# Autodesk Inventor assembly: Additional_Building
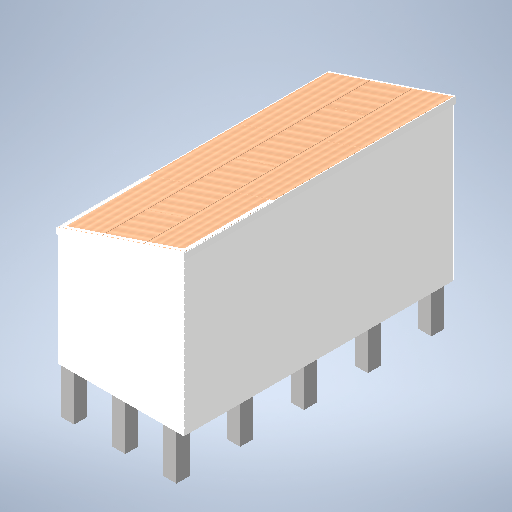
[picture p0: Inventor's stored thumbnail of the model, 512x512]
Saved by Autodesk Inventor 2025 (Build 290162010, 162A)
## iProperties
Created: 2024-08-02
Part Number: Additional_Building
Document SubType Name: Assembly
Designer: Tom
Author: Tom
## Documents named in this file (52)
- C:\Users\Tom\Documents\Inventor\Mobility\Additional_Building\Additional_Building.iam
- C:\Users\Tom\Documents\Inventor\Mobility\Additional_Building\Grid_Of_Piers.iam
- C:\Users\Tom\Documents\Inventor\Mobility\Additional_Building\Floor_System.iam
- C:\Users\Tom\Documents\Inventor\Mobility\Additional_Building\Walls.iam
- C:\Users\Tom\Documents\Inventor\Mobility\Additional_Building\Truss.iam
- C:\Users\Tom\Documents\Inventor\Mobility\Additional_Building\OSB_For_Walls_With_Dimensions_48_x_96_Inches.ipt
- C:\Users\Tom\Documents\Inventor\Mobility\Additional_Building\OSB_For_Walls_With_Dimensions_48_x_48_Inches.ipt
- C:\Users\Tom\Documents\Inventor\Mobility\Additional_Building\OSB_For_Roof_With_Dimensions_96_x_48.ipt
- C:\Users\Tom\Documents\Inventor\Mobility\Additional_Building\OSB_For_Walls_With_Dimensions_25.5_x_96_Inches.ipt
- C:\Users\Tom\Documents\Inventor\Mobility\Additional_Building\Subfascia_With_Dimensions_4.023_x_13.75_Inches.ipt
- C:\Users\Tom\Documents\Inventor\Mobility\Additional_Building\Subfascia_With_Dimensions_4.023_x_14.5_Inches.ipt
- C:\Users\Tom\Documents\Inventor\Mobility\Additional_Building\DensGlass_With_Dimensions_36.5_x_48_Inches.ipt
- C:\Users\Tom\Documents\Inventor\Mobility\Additional_Building\DensGlass_With_Dimensions_48_x_96_Inches.ipt
- C:\Users\Tom\Documents\Inventor\Mobility\Additional_Building\DensGlass_With_Dimensions_48_x_84.5_Inches.ipt
- C:\Users\Tom\Documents\Inventor\Mobility\Additional_Building\DensGlass_With_Dimensions_60.75_x_12_Inches.ipt
- C:\Users\Tom\Documents\Inventor\Mobility\Additional_Building\DensGlass_With_Dimensions_36.5_x_25.5_Inches.ipt
- C:\Users\Tom\Documents\Inventor\Mobility\Additional_Building\DensGlass_With_Dimensions_25.5_x_96_Inches.ipt
- C:\Users\Tom\Documents\Inventor\Mobility\Additional_Building\Siding_For_Back_Wall.iam
- C:\Users\Tom\Documents\Inventor\Mobility\Additional_Building\Fascia_For_Back.ipt
- C:\Users\Tom\Documents\Inventor\Mobility\Additional_Building\OSB_For_Side_And_Back.ipt
- C:\Users\Tom\Documents\Inventor\Mobility\Additional_Building\OSB_For_Roof_With_Dimensions_48_x_48.ipt
- C:\Users\Tom\Documents\Inventor\Mobility\Additional_Building\OSB_For_Roof_With_Dimensions_46.416_x_96.ipt
- C:\Users\Tom\Documents\Inventor\Mobility\Additional_Building\Stud_Between_Top_Plate_And_Rafter_1.ipt
- C:\Users\Tom\Documents\Inventor\Mobility\Additional_Building\Stud_Between_Top_Plate_And_Rafter_2.ipt
- C:\Users\Tom\Documents\Inventor\Mobility\Additional_Building\Stud_Between_Top_Plate_And_Rafter_3.ipt
- C:\Users\Tom\Documents\Inventor\Mobility\Additional_Building\Stud_Between_Top_Plate_And_Rafter_4.ipt
- C:\Users\Tom\Documents\Inventor\Mobility\Additional_Building\Stud_Between_Top_Plate_And_Rafter_5.ipt
- C:\Users\Tom\Documents\Inventor\Mobility\Additional_Building\Stud_Between_Top_Plate_And_Rafter_6.ipt
- C:\Users\Tom\Documents\Inventor\Mobility\Additional_Building\Stud_Between_Top_Plate_And_Rafter_7.ipt
- C:\Users\Tom\Documents\Inventor\Mobility\Additional_Building\Stud_Between_Top_Plate_And_Rafter_8.ipt
- C:\Users\Tom\Documents\Inventor\Mobility\Additional_Building\Stud_Between_Top_Plate_And_Rafter_9.ipt
- C:\Users\Tom\Documents\Inventor\Mobility\Additional_Building\Stud_With_Height_41.707_Inches.ipt
- C:\Users\Tom\Documents\Inventor\Mobility\Additional_Building\Support_For_Ceiling.ipt
- C:\Users\Tom\Documents\Inventor\Mobility\Additional_Building\OSB_For_Side_And_Front.ipt
- C:\Users\Tom\Documents\Inventor\Mobility\Additional_Building\OSB_For_Side_And_Top.ipt
- C:\Users\Tom\Documents\Inventor\Mobility\Additional_Building\Subfascia_With_Dimensions_5.798_x_13.75_Inches.ipt
- C:\Users\Tom\Documents\Inventor\Mobility\Additional_Building\Subfascia_With_Dimensions_5.798_x_14.5_Inches.ipt
- C:\Users\Tom\Documents\Inventor\Mobility\Additional_Building\OSB_For_Walls_With_Dimensions_20.794_x_48_Inches.ipt
- C:\Users\Tom\Documents\Inventor\Mobility\Additional_Building\OSB_For_Walls_With_Dimensions_20.794_x_96_Inches.ipt
- C:\Users\Tom\Documents\Inventor\Mobility\Additional_Building\Siding_For_Front_Wall.iam
- C:\Users\Tom\Documents\Inventor\Mobility\Additional_Building\Fascia_For_Front.ipt
- C:\Users\Tom\Documents\Inventor\Mobility\Additional_Building\OSB_For_Walls_With_Dimensions_48_x_85_Inches.ipt
- C:\Users\Tom\Documents\Inventor\Mobility\Additional_Building\OSB_For_Walls_With_Dimensions_37_x_48_Inches.ipt
- C:\Users\Tom\Documents\Inventor\Mobility\Additional_Building\Fascia_For_Side.ipt
- C:\Users\Tom\Documents\Inventor\Mobility\Additional_Building\Drip_Edge_For_Back.ipt
- C:\Users\Tom\Documents\Inventor\Mobility\Additional_Building\OSB_For_Rear_Roof.ipt
- C:\Users\Tom\Documents\Inventor\Mobility\Additional_Building\Siding_For_Left_Wall.iam
- C:\Users\Tom\Documents\Inventor\Mobility\Additional_Building\Siding_For_Right_Wall.iam
- C:\Users\Tom\Documents\Inventor\Mobility\Additional_Building\Drip_Edge_For_Front.ipt
- C:\Users\Tom\Documents\Inventor\Mobility\Additional_Building\Drip_Edge_For_Side.ipt
- C:\Users\Tom\Documents\Inventor\Mobility\Additional_Building\Underlayment_For_Side.ipt
- C:\Users\Tom\Documents\Inventor\Mobility\Additional_Building\Underlayment_For_Front.ipt
## Components (179 placed, 51 different names)
1. Grid_Of_Piers:1 [sub-assembly] — Mate:1, Flush:1, Mate:2
2. Floor_System:1 [sub-assembly] — Mate:1, Flush:1, Mate:2, Mate:3, Flush:2, Flush:3, Flush:15, Flush:16, Flush:29, Flush:30, Flush:31, Flush:33
3. Walls:1 [sub-assembly] — Mate:3, Flush:2, Flush:3, Flush:4, Flush:5, Mate:4, Flush:7, Mate:5, Mate:9, Mate:10, Flush:17, Mate:12, Mate:15, Mate:18, Mate:68, Flush:48, Flush:49, Mate:69, Flush:50, Flush:51, Mate:70, Flush:52, Flush:53, Mate:71, Flush:54, Flush:55, Mate:72, Flush:56, Flush:57, Mate:73, Flush:58, Flush:59, Mate:74, Flush:60, Flush:61, Mate:75, Flush:62, Flush:63, Mate:76, Flush:64, Mate:78, Mate:90, Mate:113, Mate:116, Mate:119, Mate:121
4. Subfascia_With_Dimensions_4.023_x_13.75_Inches:1 — Mate:21, Flush:22, Flush:23
5. Subfascia_With_Dimensions_4.023_x_13.75_Inches:2 — Flush:26, Mate:23, Flush:27, Flush:39
6. DensGlass_With_Dimensions_36.5_x_48_Inches:1 — Mate:24, Flush:28, Flush:29, Mate:26
7. DensGlass_With_Dimensions_36.5_x_48_Inches:2 — Mate:27, Mate:28, Flush:31
8. DensGlass_With_Dimensions_48_x_84.5_Inches:1 — Mate:29, Flush:32, Mate:30, Mate:32, Mate:38, Mate:41, Mate:44
9. DensGlass_With_Dimensions_48_x_96_Inches:3 — Mate:31, Mate:32, Mate:33, Mate:35
10. DensGlass_With_Dimensions_48_x_84.5_Inches:2 — Mate:34, Mate:35, Mate:36, Mate:47
11. DensGlass_With_Dimensions_36.5_x_25.5_Inches:1 — Mate:39, Mate:40, Mate:41, Mate:43
12. DensGlass_With_Dimensions_36.5_x_25.5_Inches:2 — Mate:45, Mate:46, Mate:47
13. Siding_For_Back_Wall:1 [sub-assembly] — Mate:48, Flush:34, Flush:35
14. Underlayment_For_Front:1 — Mate:146, Flush:126, Mate:147
15. Siding_For_Front_Wall:1 [sub-assembly] — Flush:93, Flush:94, Mate:108
16. Underlayment_For_Side:1 — Mate:144, Flush:122, Flush:123
17. Siding_For_Left_Wall:1 [sub-assembly] — Mate:133, Flush:117, Mate:134
18. Fascia_For_Side:1 — Mate:126, Flush:105, Flush:108, Mate:141, Mate:142
19. Underlayment_For_Side:2 — Flush:124, Mate:145, Flush:125, Flush:126
20. Siding_For_Right_Wall:1 [sub-assembly] — Mate:135, Mate:136, Flush:118
21. Fascia_For_Side:2 — Mate:127, Flush:107, Flush:108
22. Drip_Edge_For_Side:1 — Mate:140, Mate:141, Flush:120
23. Drip_Edge_For_Back:1 — Flush:109, Mate:128, Mate:137
24. Drip_Edge_For_Front:1 — Mate:138, Flush:119
25. Truss:1 [sub-assembly] — Flush:6, Mate:23, Flush:27, Mate:50, Mate:56, Mate:77, Mate:79, Flush:65, Flush:67, Flush:69, Flush:71, Flush:73, Flush:75, Flush:77, Flush:79, Flush:81, Mate:92, Mate:96, Mate:109, Flush:104, Flush:115, Mate:132, Flush:116, Mate:153
26. Truss:2 [sub-assembly] — Flush:4, Flush:5, Mate:4, Mate:20, Mate:101, Flush:91, Mate:103, Flush:92, Flush:124, Mate:147, Flush:127
27. Truss:3 [sub-assembly] — Flush:6, Flush:7, Mate:5, Flush:26, Mate:81, Mate:82, Mate:83, Mate:84, Mate:85, Mate:86, Mate:87, Mate:88, Mate:89, Mate:91, Flush:82, Mate:99, Flush:87, Flush:88
28. Truss:4 [sub-assembly] — Mate:100, Flush:89, Flush:90
29. Truss:5 [sub-assembly]
30. Truss:6 [sub-assembly]
31. Truss:7 [sub-assembly]
32. Truss:8 [sub-assembly]
33. Truss:9 [sub-assembly]
34. Truss:10 [sub-assembly]
35. Truss:11 [sub-assembly]
36. Truss:12 [sub-assembly]
37. Truss:13 [sub-assembly]
38. Truss:14 [sub-assembly]
39. Truss:15 [sub-assembly] — Mate:63
40. Truss:16 [sub-assembly] — Mate:105
41. Truss:17 [sub-assembly]
42. Truss:18 [sub-assembly] — Mate:22, Flush:25
43. Truss:19 [sub-assembly] — Mate:21, Flush:22, Flush:23, Flush:24, Mate:149
44. OSB_For_Walls_With_Dimensions_25.5_x_96_Inches:1 — Mate:18, Flush:18, Mate:20, Mate:39
45. OSB_For_Walls_With_Dimensions_25.5_x_96_Inches:2 — Mate:42
46. OSB_For_Walls_With_Dimensions_25.5_x_96_Inches:3 — Mate:45
47. OSB_For_Walls_With_Dimensions_48_x_48_Inches:2 — Mate:15, Mate:16, Mate:17, Mate:29, Flush:32
48. OSB_For_Walls_With_Dimensions_48_x_48_Inches:1 — Mate:10, Mate:11, Flush:17, Mate:13, Mate:34
49. OSB_For_Walls_With_Dimensions_48_x_48_Inches:3 — Mate:102
50. OSB_For_Walls_With_Dimensions_48_x_48_Inches:4
51. OSB_For_Walls_With_Dimensions_48_x_96_Inches:13 — Mate:101, Mate:102, Flush:91, Mate:104, Mate:108
52. OSB_For_Walls_With_Dimensions_48_x_96_Inches:14 — Mate:106
53. OSB_For_Walls_With_Dimensions_48_x_96_Inches:15 — Mate:146
54. OSB_For_Walls_With_Dimensions_20.794_x_96_Inches:1 — Mate:105, Mate:106, Mate:107
55. OSB_For_Walls_With_Dimensions_20.794_x_96_Inches:2
56. OSB_For_Walls_With_Dimensions_20.794_x_48_Inches:1 — Mate:103, Mate:104, Flush:92, Mate:107
57. OSB_For_Walls_With_Dimensions_20.794_x_48_Inches:2
58. Subfascia_With_Dimensions_4.023_x_14.5_Inches:1 — Flush:24, Mate:22, Flush:25
59. Subfascia_With_Dimensions_4.023_x_14.5_Inches:2
60. Subfascia_With_Dimensions_4.023_x_14.5_Inches:3
61. Subfascia_With_Dimensions_4.023_x_14.5_Inches:4
62. Subfascia_With_Dimensions_4.023_x_14.5_Inches:5
63. Subfascia_With_Dimensions_4.023_x_14.5_Inches:6
64. Subfascia_With_Dimensions_4.023_x_14.5_Inches:7
65. Subfascia_With_Dimensions_4.023_x_14.5_Inches:8
66. Subfascia_With_Dimensions_4.023_x_14.5_Inches:9
67. Subfascia_With_Dimensions_4.023_x_14.5_Inches:10
68. Subfascia_With_Dimensions_4.023_x_14.5_Inches:11
69. Subfascia_With_Dimensions_4.023_x_14.5_Inches:12
70. Subfascia_With_Dimensions_4.023_x_14.5_Inches:13
71. Subfascia_With_Dimensions_4.023_x_14.5_Inches:14
72. Subfascia_With_Dimensions_4.023_x_14.5_Inches:15
73. Subfascia_With_Dimensions_4.023_x_14.5_Inches:16
74. DensGlass_With_Dimensions_48_x_96_Inches:1 — Mate:25, Mate:26, Flush:30, Mate:30, Mate:33
75. DensGlass_With_Dimensions_48_x_96_Inches:2 — Mate:28, Mate:36
76. DensGlass_With_Dimensions_60.75_x_12_Inches:1 — Mate:37, Mate:38, Flush:33
77. DensGlass_With_Dimensions_60.75_x_12_Inches:2 — Mate:48, Flush:34, Flush:35
78. DensGlass_With_Dimensions_60.75_x_12_Inches:3 — Mate:40
79. DensGlass_With_Dimensions_60.75_x_12_Inches:4 — Mate:57, Mate:115
80. DensGlass_With_Dimensions_25.5_x_96_Inches:1 — Mate:42, Mate:43, Mate:44
81. DensGlass_With_Dimensions_25.5_x_96_Inches:2 — Mate:46
82. Stud_Between_Top_Plate_And_Rafter_1:1 — Mate:68, Flush:48, Flush:49, Flush:66
83. Stud_Between_Top_Plate_And_Rafter_2:1 — Mate:69, Flush:50, Flush:51, Flush:68
84. Stud_Between_Top_Plate_And_Rafter_3:1 — Mate:70, Flush:52, Flush:53, Flush:70
85. Stud_Between_Top_Plate_And_Rafter_4:1 — Mate:71, Flush:54, Flush:55, Flush:72
86. Stud_Between_Top_Plate_And_Rafter_5:1 — Mate:72, Flush:56, Flush:57, Flush:74
87. Stud_Between_Top_Plate_And_Rafter_6:1 — Mate:73, Flush:58, Flush:59, Flush:76
88. Stud_Between_Top_Plate_And_Rafter_7:1 — Mate:74, Flush:60, Flush:61, Flush:78
89. Stud_Between_Top_Plate_And_Rafter_9:1 — Mate:76, Mate:77, Flush:64, Mate:80
90. Stud_Between_Top_Plate_And_Rafter_8:1 — Mate:75, Flush:62, Flush:63, Flush:80
91. Stud_Between_Top_Plate_And_Rafter_1:2
92. Stud_Between_Top_Plate_And_Rafter_2:2
93. Stud_Between_Top_Plate_And_Rafter_3:2
94. Stud_Between_Top_Plate_And_Rafter_4:2
95. Stud_Between_Top_Plate_And_Rafter_5:2
96. Stud_Between_Top_Plate_And_Rafter_6:2
97. Stud_Between_Top_Plate_And_Rafter_7:2
98. Stud_Between_Top_Plate_And_Rafter_9:2
99. Stud_Between_Top_Plate_And_Rafter_8:2
100. Stud_With_Height_41.707_Inches:1 — Mate:78, Mate:79, Mate:80
101. Stud_With_Height_41.707_Inches:2
102. Support_For_Ceiling:9 — Mate:89, Flush:81, Mate:90
103. Support_For_Ceiling:1 — Mate:81, Flush:65, Flush:66
104. Support_For_Ceiling:2 — Mate:82, Flush:67, Flush:68
105. Support_For_Ceiling:3 — Mate:83, Flush:69, Flush:70
106. Support_For_Ceiling:4 — Mate:84, Flush:71, Flush:72
107. Support_For_Ceiling:5 — Mate:85, Flush:73, Flush:74
108. Support_For_Ceiling:6 — Mate:86, Flush:75, Flush:76
109. Support_For_Ceiling:7 — Mate:87, Flush:77, Flush:78
110. Support_For_Ceiling:8 — Mate:88, Flush:79, Flush:80
111. Support_For_Ceiling:10 — Mate:91, Flush:82, Mate:92
112. Support_For_Ceiling:11
113. Support_For_Ceiling:12
114. Support_For_Ceiling:13
115. Support_For_Ceiling:14
116. Support_For_Ceiling:15
117. Support_For_Ceiling:16
118. Support_For_Ceiling:17
119. Support_For_Ceiling:18
120. Support_For_Ceiling:19
121. Support_For_Ceiling:20
122. Subfascia_With_Dimensions_5.798_x_13.75_Inches:1 — Mate:99, Flush:87, Flush:88
123. Subfascia_With_Dimensions_5.798_x_13.75_Inches:2
124. Subfascia_With_Dimensions_5.798_x_14.5_Inches:1 — Mate:100, Flush:89, Flush:90
125. Subfascia_With_Dimensions_5.798_x_14.5_Inches:2
126. Subfascia_With_Dimensions_5.798_x_14.5_Inches:3
127. Subfascia_With_Dimensions_5.798_x_14.5_Inches:4
128. Subfascia_With_Dimensions_5.798_x_14.5_Inches:5
129. Subfascia_With_Dimensions_5.798_x_14.5_Inches:6
130. Subfascia_With_Dimensions_5.798_x_14.5_Inches:7
131. Subfascia_With_Dimensions_5.798_x_14.5_Inches:8
132. Subfascia_With_Dimensions_5.798_x_14.5_Inches:9
133. Subfascia_With_Dimensions_5.798_x_14.5_Inches:10
134. Subfascia_With_Dimensions_5.798_x_14.5_Inches:11
135. Subfascia_With_Dimensions_5.798_x_14.5_Inches:12
136. Subfascia_With_Dimensions_5.798_x_14.5_Inches:13
137. Subfascia_With_Dimensions_5.798_x_14.5_Inches:14
138. Subfascia_With_Dimensions_5.798_x_14.5_Inches:15
139. Subfascia_With_Dimensions_5.798_x_14.5_Inches:16
140. Fascia_For_Back:1 — Mate:50, Flush:39, Flush:104, Flush:105, Flush:109, Mate:128, Mate:134, Mate:142
141. Fascia_For_Back:2
142. Fascia_For_Back:3 — Mate:136
143. Fascia_For_Front:1 — Mate:109, Flush:95, Flush:96, Mate:126, Mate:138, Flush:119
144. Fascia_For_Front:2
145. Fascia_For_Front:3 — Mate:127, Flush:107
146. OSB_For_Walls_With_Dimensions_48_x_96_Inches:16 — Mate:119, Mate:120, Flush:98, Mate:131, Mate:133, Flush:117
147. OSB_For_Walls_With_Dimensions_37_x_48_Inches:1 — Mate:121, Mate:122, Mate:131, Flush:122
148. OSB_For_Walls_With_Dimensions_48_x_48_Inches:5 — Mate:113, Mate:114, Mate:115, Mate:117, Mate:120
149. OSB_For_Walls_With_Dimensions_48_x_85_Inches:1 — Mate:116, Mate:117, Mate:118, Mate:122
150. OSB_For_Side_And_Back:1 — Mate:56, Mate:57, Flush:83, Mate:98, Mate:111, Mate:112, Mate:114, Mate:118, Flush:128
151. OSB_For_Side_And_Front:1 — Flush:83, Mate:97, Mate:111, Mate:112, Flush:97
152. OSB_For_Side_And_Top:1 — Mate:96, Mate:97, Flush:95, Flush:96, Flush:97, Mate:144, Flush:123
153. OSB_For_Walls_With_Dimensions_48_x_96_Inches:17 — Mate:135
154. OSB_For_Walls_With_Dimensions_37_x_48_Inches:2 — Flush:118
155. OSB_For_Walls_With_Dimensions_48_x_48_Inches:6
156. OSB_For_Walls_With_Dimensions_48_x_85_Inches:2
157. OSB_For_Side_And_Back:2
158. OSB_For_Side_And_Front:2
159. OSB_For_Side_And_Top:2 — Mate:145, Mate:148
160. OSB_For_Rear_Roof:1 — Flush:115, Mate:132, Flush:116, Mate:140, Flush:120, Flush:128
161. OSB_For_Rear_Roof:2 — Mate:137
162. OSB_For_Rear_Roof:3 — Mate:150, Mate:151
163. OSB_For_Roof_With_Dimensions_48_x_48:1 — Mate:65, Mate:148, Mate:149, Mate:150, Mate:152
164. OSB_For_Roof_With_Dimensions_48_x_48:2
165. OSB_For_Roof_With_Dimensions_96_x_48:4 — Mate:63, Mate:65, Mate:151
166. OSB_For_Roof_With_Dimensions_96_x_48:5
167. OSB_For_Roof_With_Dimensions_46.416_x_96:1 — Mate:152, Mate:153, Flush:127
168. OSB_For_Roof_With_Dimensions_46.416_x_96:2
169. OSB_For_Roof_With_Dimensions_46.416_x_96:3
170. OSB_For_Walls_With_Dimensions_48_x_96_Inches:1 — Mate:9, Flush:15, Flush:16, Mate:11, Mate:16, Flush:18, Mate:24, Flush:28, Mate:25, Mate:37
171. OSB_For_Walls_With_Dimensions_48_x_96_Inches:2
172. OSB_For_Walls_With_Dimensions_48_x_96_Inches:3 — Mate:14, Mate:27, Flush:98
173. OSB_For_Walls_With_Dimensions_48_x_96_Inches:4 — Mate:12, Mate:13, Mate:14, Mate:31
174. OSB_For_Walls_With_Dimensions_48_x_96_Inches:5 — Mate:17
175. OSB_For_Walls_With_Dimensions_48_x_96_Inches:8 — Flush:93, Flush:94, Flush:125
176. OSB_For_Walls_With_Dimensions_48_x_96_Inches:9
177. OSB_For_Walls_With_Dimensions_48_x_96_Inches:10
178. OSB_For_Walls_With_Dimensions_48_x_96_Inches:11
179. OSB_For_Walls_With_Dimensions_48_x_96_Inches:12
## Component patterns: (2 elements, first: Truss:1), (17 elements, first: Truss:3), (3 elements, first: OSB_For_Walls_With_Dimensions_25.5_x_96_Inches:1), (2 elements, first: OSB_For_Walls_With_Dimensions_48_x_48_Inches:2 + OSB_For_Walls_With_Dimensions_48_x_48_Inches:1), (3 elements, first: OSB_For_Walls_With_Dimensions_48_x_96_Inches:13), (2 elements, first: OSB_For_Walls_With_Dimensions_20.794_x_96_Inches:1), (2 elements, first: OSB_For_Walls_With_Dimensions_20.794_x_48_Inches:1), (16 elements, first: Subfascia_With_Dimensions_4.023_x_14.5_Inches:1), (2 elements, first: DensGlass_With_Dimensions_48_x_96_Inches:1), (4 elements, first: DensGlass_With_Dimensions_60.75_x_12_Inches:1), (2 elements, first: DensGlass_With_Dimensions_25.5_x_96_Inches:1), (2 elements, first: Stud_Between_Top_Plate_And_Rafter_1:1 + Stud_Between_Top_Plate_And_Rafter_2:1 + Stud_Between_Top_Plate_And_Rafter_3:1 + Stud_Between_Top_Plate_And_Rafter_4:1 + Stud_Between_Top_Plate_And_Rafter_5:1 + Stud_Between_Top_Plate_And_Rafter_6:1 + Stud_Between_Top_Plate_And_Rafter_7:1 + Stud_Between_Top_Plate_And_Rafter_9:1 + Stud_Between_Top_Plate_And_Rafter_8:1), (2 elements, first: Stud_With_Height_41.707_Inches:1), (2 elements, first: Support_For_Ceiling:9 + Support_For_Ceiling:1 + Support_For_Ceiling:2 + Support_For_Ceiling:3 + Support_For_Ceiling:4 + Support_For_Ceiling:5 + Support_For_Ceiling:6 + Support_For_Ceiling:7 + Support_For_Ceiling:8 + Support_For_Ceiling:10), (2 elements, first: Subfascia_With_Dimensions_5.798_x_13.75_Inches:1), (16 elements, first: Subfascia_With_Dimensions_5.798_x_14.5_Inches:1), (3 elements, first: Fascia_For_Back:1), (3 elements, first: Fascia_For_Front:1), (2 elements, first: OSB_For_Walls_With_Dimensions_48_x_96_Inches:16 + OSB_For_Walls_With_Dimensions_37_x_48_Inches:1 + OSB_For_Walls_With_Dimensions_48_x_48_Inches:5 + OSB_For_Walls_With_Dimensions_48_x_85_Inches:1 + OSB_For_Side_And_Back:1 + OSB_For_Side_And_Front:1 + OSB_For_Side_And_Top:1), (3 elements, first: OSB_For_Rear_Roof:1), (2 elements, first: OSB_For_Roof_With_Dimensions_48_x_48:1), (2 elements, first: OSB_For_Roof_With_Dimensions_96_x_48:4), (3 elements, first: OSB_For_Roof_With_Dimensions_46.416_x_96:1), (3 elements, first: OSB_For_Walls_With_Dimensions_48_x_96_Inches:1), (2 elements, first: OSB_For_Walls_With_Dimensions_48_x_96_Inches:4), Component Pattern 3:2 (3 elements), Component Pattern 4:2 (2 elements)
## Relationships (217: Mate 124, Flush 92, Angle 1)
- Mate:1: Grid_Of_Piers:1 ↔ Floor_System:1
- Flush:1: Grid_Of_Piers:1 ↔ Floor_System:1
- Mate:2: Grid_Of_Piers:1 ↔ Floor_System:1
- Mate:3: Floor_System:1 ↔ Walls:1
- Flush:2: Floor_System:1 ↔ Walls:1
- Flush:3: Floor_System:1 ↔ Walls:1
- Flush:4: Walls:1 ↔ Truss:2
- Flush:5: Walls:1 ↔ Truss:2
- Mate:4: Walls:1 ↔ Truss:2
- Flush:6 (387.35 mm): Truss:1 ↔ Truss:3
- Flush:7: Walls:1 ↔ Truss:3
- Mate:5: Walls:1 ↔ Truss:3
- Mate:9: Walls:1 ↔ OSB_For_Walls_With_Dimensions_48_x_96_Inches:1
- Flush:15: Floor_System:1 ↔ OSB_For_Walls_With_Dimensions_48_x_96_Inches:1
- Flush:16: Floor_System:1 ↔ OSB_For_Walls_With_Dimensions_48_x_96_Inches:1
- Mate:10: Walls:1 ↔ OSB_For_Walls_With_Dimensions_48_x_48_Inches:1
- Mate:11: OSB_For_Walls_With_Dimensions_48_x_48_Inches:1 ↔ OSB_For_Walls_With_Dimensions_48_x_96_Inches:1
- Flush:17: Walls:1 ↔ OSB_For_Walls_With_Dimensions_48_x_48_Inches:1
- Mate:12: Walls:1 ↔ OSB_For_Walls_With_Dimensions_48_x_96_Inches:4
- Mate:13: OSB_For_Walls_With_Dimensions_48_x_48_Inches:1 ↔ OSB_For_Walls_With_Dimensions_48_x_96_Inches:4
- Mate:14: OSB_For_Walls_With_Dimensions_48_x_96_Inches:3 ↔ OSB_For_Walls_With_Dimensions_48_x_96_Inches:4
- Mate:15: Walls:1 ↔ OSB_For_Walls_With_Dimensions_48_x_48_Inches:2
- Mate:16: OSB_For_Walls_With_Dimensions_48_x_48_Inches:2 ↔ OSB_For_Walls_With_Dimensions_48_x_96_Inches:1
- Mate:17: OSB_For_Walls_With_Dimensions_48_x_48_Inches:2 ↔ OSB_For_Walls_With_Dimensions_48_x_96_Inches:5
- Mate:18: Walls:1 ↔ OSB_For_Walls_With_Dimensions_25.5_x_96_Inches:1
- Flush:18: OSB_For_Walls_With_Dimensions_25.5_x_96_Inches:1 ↔ OSB_For_Walls_With_Dimensions_48_x_96_Inches:1
- Mate:20: Truss:2 ↔ OSB_For_Walls_With_Dimensions_25.5_x_96_Inches:1
- Mate:21: Subfascia_With_Dimensions_4.023_x_13.75_Inches:1 ↔ Truss:19
- Flush:22: Subfascia_With_Dimensions_4.023_x_13.75_Inches:1 ↔ Truss:19
- Flush:23: Subfascia_With_Dimensions_4.023_x_13.75_Inches:1 ↔ Truss:19
- Flush:24: Truss:19 ↔ Subfascia_With_Dimensions_4.023_x_14.5_Inches:1
- Mate:22: Truss:18 ↔ Subfascia_With_Dimensions_4.023_x_14.5_Inches:1
- Flush:25: Truss:18 ↔ Subfascia_With_Dimensions_4.023_x_14.5_Inches:1
- Flush:26: Subfascia_With_Dimensions_4.023_x_13.75_Inches:2 ↔ Truss:3
- Mate:23: Subfascia_With_Dimensions_4.023_x_13.75_Inches:2 ↔ Truss:1
- Flush:27: Subfascia_With_Dimensions_4.023_x_13.75_Inches:2 ↔ Truss:1
- Mate:24: DensGlass_With_Dimensions_36.5_x_48_Inches:1 ↔ OSB_For_Walls_With_Dimensions_48_x_96_Inches:1
- Flush:28 (292.1 mm): DensGlass_With_Dimensions_36.5_x_48_Inches:1 ↔ OSB_For_Walls_With_Dimensions_48_x_96_Inches:1
- Flush:29: Floor_System:1 ↔ DensGlass_With_Dimensions_36.5_x_48_Inches:1
- Mate:25: DensGlass_With_Dimensions_48_x_96_Inches:1 ↔ OSB_For_Walls_With_Dimensions_48_x_96_Inches:1
- Mate:26: DensGlass_With_Dimensions_36.5_x_48_Inches:1 ↔ DensGlass_With_Dimensions_48_x_96_Inches:1
- Flush:30: Floor_System:1 ↔ DensGlass_With_Dimensions_48_x_96_Inches:1
- Mate:27: DensGlass_With_Dimensions_36.5_x_48_Inches:2 ↔ OSB_For_Walls_With_Dimensions_48_x_96_Inches:3
- Mate:28: DensGlass_With_Dimensions_36.5_x_48_Inches:2 ↔ DensGlass_With_Dimensions_48_x_96_Inches:2
- Flush:31: Floor_System:1 ↔ DensGlass_With_Dimensions_36.5_x_48_Inches:2
- Mate:29: DensGlass_With_Dimensions_48_x_84.5_Inches:1 ↔ OSB_For_Walls_With_Dimensions_48_x_48_Inches:2
- Flush:32 (292.1 mm): DensGlass_With_Dimensions_48_x_84.5_Inches:1 ↔ OSB_For_Walls_With_Dimensions_48_x_48_Inches:2
- Mate:30: DensGlass_With_Dimensions_48_x_84.5_Inches:1 ↔ DensGlass_With_Dimensions_48_x_96_Inches:1
- Mate:31: DensGlass_With_Dimensions_48_x_96_Inches:3 ↔ OSB_For_Walls_With_Dimensions_48_x_96_Inches:4
- Mate:32: DensGlass_With_Dimensions_48_x_84.5_Inches:1 ↔ DensGlass_With_Dimensions_48_x_96_Inches:3
- Mate:33: DensGlass_With_Dimensions_48_x_96_Inches:3 ↔ DensGlass_With_Dimensions_48_x_96_Inches:1
- Mate:34: DensGlass_With_Dimensions_48_x_84.5_Inches:2 ↔ OSB_For_Walls_With_Dimensions_48_x_48_Inches:1
- Mate:35: DensGlass_With_Dimensions_48_x_96_Inches:3 ↔ DensGlass_With_Dimensions_48_x_84.5_Inches:2
- Mate:36: DensGlass_With_Dimensions_48_x_84.5_Inches:2 ↔ DensGlass_With_Dimensions_48_x_96_Inches:2
- Mate:37: DensGlass_With_Dimensions_60.75_x_12_Inches:1 ↔ OSB_For_Walls_With_Dimensions_48_x_96_Inches:1
- Mate:38: DensGlass_With_Dimensions_48_x_84.5_Inches:1 ↔ DensGlass_With_Dimensions_60.75_x_12_Inches:1
- Flush:33: Floor_System:1 ↔ DensGlass_With_Dimensions_60.75_x_12_Inches:1
- Mate:39: DensGlass_With_Dimensions_36.5_x_25.5_Inches:1 ↔ OSB_For_Walls_With_Dimensions_25.5_x_96_Inches:1
- Mate:40: DensGlass_With_Dimensions_36.5_x_25.5_Inches:1 ↔ DensGlass_With_Dimensions_60.75_x_12_Inches:3
- Mate:41: DensGlass_With_Dimensions_48_x_84.5_Inches:1 ↔ DensGlass_With_Dimensions_36.5_x_25.5_Inches:1
- Mate:42: OSB_For_Walls_With_Dimensions_25.5_x_96_Inches:2 ↔ DensGlass_With_Dimensions_25.5_x_96_Inches:1
- Mate:43: DensGlass_With_Dimensions_36.5_x_25.5_Inches:1 ↔ DensGlass_With_Dimensions_25.5_x_96_Inches:1
- Mate:44: DensGlass_With_Dimensions_48_x_84.5_Inches:1 ↔ DensGlass_With_Dimensions_25.5_x_96_Inches:1
- Mate:45: DensGlass_With_Dimensions_36.5_x_25.5_Inches:2 ↔ OSB_For_Walls_With_Dimensions_25.5_x_96_Inches:3
- Mate:46: DensGlass_With_Dimensions_36.5_x_25.5_Inches:2 ↔ DensGlass_With_Dimensions_25.5_x_96_Inches:2
- Mate:47: DensGlass_With_Dimensions_48_x_84.5_Inches:2 ↔ DensGlass_With_Dimensions_36.5_x_25.5_Inches:2
- Mate:48: Siding_For_Back_Wall:1 ↔ DensGlass_With_Dimensions_60.75_x_12_Inches:2
- Flush:34: Siding_For_Back_Wall:1 ↔ DensGlass_With_Dimensions_60.75_x_12_Inches:2
- Flush:35: Siding_For_Back_Wall:1 ↔ DensGlass_With_Dimensions_60.75_x_12_Inches:2
- Mate:50: Truss:1 ↔ Fascia_For_Back:1
- Flush:39 (-29.3688 mm): Subfascia_With_Dimensions_4.023_x_13.75_Inches:2 ↔ Fascia_For_Back:1
- Mate:56: Truss:1 ↔ OSB_For_Side_And_Back:1
- Mate:57: DensGlass_With_Dimensions_60.75_x_12_Inches:4 ↔ OSB_For_Side_And_Back:1
- Mate:63: Truss:15 ↔ OSB_For_Roof_With_Dimensions_96_x_48:4
- Mate:65: OSB_For_Roof_With_Dimensions_48_x_48:1 ↔ OSB_For_Roof_With_Dimensions_96_x_48:4
- Mate:68: Walls:1 ↔ Stud_Between_Top_Plate_And_Rafter_1:1
- Flush:48: Walls:1 ↔ Stud_Between_Top_Plate_And_Rafter_1:1
- Flush:49: Walls:1 ↔ Stud_Between_Top_Plate_And_Rafter_1:1
- Mate:69: Walls:1 ↔ Stud_Between_Top_Plate_And_Rafter_2:1
- Flush:50: Walls:1 ↔ Stud_Between_Top_Plate_And_Rafter_2:1
- Flush:51: Walls:1 ↔ Stud_Between_Top_Plate_And_Rafter_2:1
- Mate:70: Walls:1 ↔ Stud_Between_Top_Plate_And_Rafter_3:1
- Flush:52: Walls:1 ↔ Stud_Between_Top_Plate_And_Rafter_3:1
- Flush:53: Walls:1 ↔ Stud_Between_Top_Plate_And_Rafter_3:1
- Mate:71: Walls:1 ↔ Stud_Between_Top_Plate_And_Rafter_4:1
- Flush:54: Walls:1 ↔ Stud_Between_Top_Plate_And_Rafter_4:1
- Flush:55: Walls:1 ↔ Stud_Between_Top_Plate_And_Rafter_4:1
- Mate:72: Walls:1 ↔ Stud_Between_Top_Plate_And_Rafter_5:1
- Flush:56: Walls:1 ↔ Stud_Between_Top_Plate_And_Rafter_5:1
- Flush:57: Walls:1 ↔ Stud_Between_Top_Plate_And_Rafter_5:1
- Mate:73: Walls:1 ↔ Stud_Between_Top_Plate_And_Rafter_6:1
- Flush:58: Walls:1 ↔ Stud_Between_Top_Plate_And_Rafter_6:1
- Flush:59: Walls:1 ↔ Stud_Between_Top_Plate_And_Rafter_6:1
- Mate:74: Walls:1 ↔ Stud_Between_Top_Plate_And_Rafter_7:1
- Flush:60: Walls:1 ↔ Stud_Between_Top_Plate_And_Rafter_7:1
- Flush:61: Walls:1 ↔ Stud_Between_Top_Plate_And_Rafter_7:1
- Mate:75: Walls:1 ↔ Stud_Between_Top_Plate_And_Rafter_8:1
- Flush:62: Walls:1 ↔ Stud_Between_Top_Plate_And_Rafter_8:1
- Flush:63: Walls:1 ↔ Stud_Between_Top_Plate_And_Rafter_8:1
- Mate:76: Walls:1 ↔ Stud_Between_Top_Plate_And_Rafter_9:1
- Mate:77: Truss:1 ↔ Stud_Between_Top_Plate_And_Rafter_9:1
- Flush:64: Walls:1 ↔ Stud_Between_Top_Plate_And_Rafter_9:1
- Mate:78: Walls:1 ↔ Stud_With_Height_41.707_Inches:1
- Mate:79: Truss:1 ↔ Stud_With_Height_41.707_Inches:1
- Mate:80: Stud_Between_Top_Plate_And_Rafter_9:1 ↔ Stud_With_Height_41.707_Inches:1
- Mate:81: Truss:3 ↔ Support_For_Ceiling:1
- Flush:65: Truss:1 ↔ Support_For_Ceiling:1
- Flush:66: Stud_Between_Top_Plate_And_Rafter_1:1 ↔ Support_For_Ceiling:1
- Mate:82: Truss:3 ↔ Support_For_Ceiling:2
- Flush:67: Truss:1 ↔ Support_For_Ceiling:2
- Flush:68: Stud_Between_Top_Plate_And_Rafter_2:1 ↔ Support_For_Ceiling:2
- Mate:83: Truss:3 ↔ Support_For_Ceiling:3
- Flush:69: Truss:1 ↔ Support_For_Ceiling:3
- Flush:70: Stud_Between_Top_Plate_And_Rafter_3:1 ↔ Support_For_Ceiling:3
- Mate:84: Truss:3 ↔ Support_For_Ceiling:4
- Flush:71: Truss:1 ↔ Support_For_Ceiling:4
- Flush:72: Stud_Between_Top_Plate_And_Rafter_4:1 ↔ Support_For_Ceiling:4
- Mate:85: Truss:3 ↔ Support_For_Ceiling:5
- Flush:73: Truss:1 ↔ Support_For_Ceiling:5
- Flush:74: Stud_Between_Top_Plate_And_Rafter_5:1 ↔ Support_For_Ceiling:5
- Mate:86: Truss:3 ↔ Support_For_Ceiling:6
- Flush:75: Truss:1 ↔ Support_For_Ceiling:6
- Flush:76: Stud_Between_Top_Plate_And_Rafter_6:1 ↔ Support_For_Ceiling:6
- Mate:87: Truss:3 ↔ Support_For_Ceiling:7
- Flush:77: Truss:1 ↔ Support_For_Ceiling:7
- Flush:78: Stud_Between_Top_Plate_And_Rafter_7:1 ↔ Support_For_Ceiling:7
- Mate:88: Truss:3 ↔ Support_For_Ceiling:8
- Flush:79: Truss:1 ↔ Support_For_Ceiling:8
- Flush:80: Stud_Between_Top_Plate_And_Rafter_8:1 ↔ Support_For_Ceiling:8
- Mate:89: Truss:3 ↔ Support_For_Ceiling:9
- Flush:81: Truss:1 ↔ Support_For_Ceiling:9
- Mate:90: Walls:1 ↔ Support_For_Ceiling:9
- Mate:91: Truss:3 ↔ Support_For_Ceiling:10
- Flush:82: Truss:3 ↔ Support_For_Ceiling:10
- Mate:92: Truss:1 ↔ Support_For_Ceiling:10
- Flush:83: OSB_For_Side_And_Back:1 ↔ OSB_For_Side_And_Front:1
- Mate:96: Truss:1 ↔ OSB_For_Side_And_Top:1
- Mate:97: OSB_For_Side_And_Front:1 ↔ OSB_For_Side_And_Top:1
- Mate:98: OSB_For_Side_And_Back:1
- Angle:1 (0 deg)
- Mate:99: Truss:3 ↔ Subfascia_With_Dimensions_5.798_x_13.75_Inches:1
- Flush:87: Truss:3 ↔ Subfascia_With_Dimensions_5.798_x_13.75_Inches:1
- Flush:88: Truss:3 ↔ Subfascia_With_Dimensions_5.798_x_13.75_Inches:1
- Mate:100: Truss:4 ↔ Subfascia_With_Dimensions_5.798_x_14.5_Inches:1
- Flush:89: Truss:4 ↔ Subfascia_With_Dimensions_5.798_x_14.5_Inches:1
- Flush:90: Truss:4 ↔ Subfascia_With_Dimensions_5.798_x_14.5_Inches:1
- Mate:101: Truss:2 ↔ OSB_For_Walls_With_Dimensions_48_x_96_Inches:13
- Mate:102: OSB_For_Walls_With_Dimensions_48_x_48_Inches:3 ↔ OSB_For_Walls_With_Dimensions_48_x_96_Inches:13
- Flush:91: Truss:2 ↔ OSB_For_Walls_With_Dimensions_48_x_96_Inches:13
- Mate:103: Truss:2 ↔ OSB_For_Walls_With_Dimensions_20.794_x_48_Inches:1
- Mate:104: OSB_For_Walls_With_Dimensions_48_x_96_Inches:13 ↔ OSB_For_Walls_With_Dimensions_20.794_x_48_Inches:1
- Flush:92: Truss:2 ↔ OSB_For_Walls_With_Dimensions_20.794_x_48_Inches:1
- Mate:105: Truss:16 ↔ OSB_For_Walls_With_Dimensions_20.794_x_96_Inches:1
- Mate:106: OSB_For_Walls_With_Dimensions_48_x_96_Inches:14 ↔ OSB_For_Walls_With_Dimensions_20.794_x_96_Inches:1
- Mate:107: OSB_For_Walls_With_Dimensions_20.794_x_96_Inches:1 ↔ OSB_For_Walls_With_Dimensions_20.794_x_48_Inches:1
- Flush:93 (-6.35 mm): Siding_For_Front_Wall:1 ↔ OSB_For_Walls_With_Dimensions_48_x_96_Inches:8
- Flush:94 (-12.7 mm): Siding_For_Front_Wall:1 ↔ OSB_For_Walls_With_Dimensions_48_x_96_Inches:8
- Mate:108: Siding_For_Front_Wall:1 ↔ OSB_For_Walls_With_Dimensions_48_x_96_Inches:13
- Mate:109: Truss:1 ↔ Fascia_For_Front:1
- Flush:95 (-20.1549 mm): Fascia_For_Front:1 ↔ OSB_For_Side_And_Top:1
- Flush:96 (-44.6151 mm): Fascia_For_Front:1 ↔ OSB_For_Side_And_Top:1
- Mate:111: OSB_For_Side_And_Back:1 ↔ OSB_For_Side_And_Front:1
- Mate:112: OSB_For_Side_And_Back:1 ↔ OSB_For_Side_And_Front:1
- Flush:97: OSB_For_Side_And_Front:1 ↔ OSB_For_Side_And_Top:1
- Mate:113: Walls:1 ↔ OSB_For_Walls_With_Dimensions_48_x_48_Inches:5
- Mate:114: OSB_For_Walls_With_Dimensions_48_x_48_Inches:5 ↔ OSB_For_Side_And_Back:1
- Mate:115: DensGlass_With_Dimensions_60.75_x_12_Inches:4 ↔ OSB_For_Walls_With_Dimensions_48_x_48_Inches:5
- Mate:116: Walls:1 ↔ OSB_For_Walls_With_Dimensions_48_x_85_Inches:1
- Mate:117: OSB_For_Walls_With_Dimensions_48_x_48_Inches:5 ↔ OSB_For_Walls_With_Dimensions_48_x_85_Inches:1
- Mate:118: OSB_For_Walls_With_Dimensions_48_x_85_Inches:1 ↔ OSB_For_Side_And_Back:1
- Mate:119: Walls:1 ↔ OSB_For_Walls_With_Dimensions_48_x_96_Inches:16
- Mate:120: OSB_For_Walls_With_Dimensions_48_x_96_Inches:16 ↔ OSB_For_Walls_With_Dimensions_48_x_48_Inches:5
- Flush:98: OSB_For_Walls_With_Dimensions_48_x_96_Inches:16 ↔ OSB_For_Walls_With_Dimensions_48_x_96_Inches:3
- Mate:121: Walls:1 ↔ OSB_For_Walls_With_Dimensions_37_x_48_Inches:1
- Mate:122: OSB_For_Walls_With_Dimensions_37_x_48_Inches:1 ↔ OSB_For_Walls_With_Dimensions_48_x_85_Inches:1
- Mate:126: Fascia_For_Side:1 ↔ Fascia_For_Front:1
- Flush:104 (-57.3151 mm): Truss:1 ↔ Fascia_For_Back:1
- Flush:105: Fascia_For_Side:1 ↔ Fascia_For_Back:1
- Mate:127: Fascia_For_Side:2 ↔ Fascia_For_Front:3
- Flush:107: Fascia_For_Side:2 ↔ Fascia_For_Front:3
- Flush:108: Fascia_For_Side:1 ↔ Fascia_For_Side:2
- Flush:109 (-12.7 mm): Drip_Edge_For_Back:1 ↔ Fascia_For_Back:1
- Mate:128: Drip_Edge_For_Back:1 ↔ Fascia_For_Back:1
- Mate:131: OSB_For_Walls_With_Dimensions_48_x_96_Inches:16 ↔ OSB_For_Walls_With_Dimensions_37_x_48_Inches:1
- Flush:115: Truss:1 ↔ OSB_For_Rear_Roof:1
- Mate:132: Truss:1 ↔ OSB_For_Rear_Roof:1
- Flush:116: Truss:1 ↔ OSB_For_Rear_Roof:1
- Mate:133 (1.5875 mm): Siding_For_Left_Wall:1 ↔ OSB_For_Walls_With_Dimensions_48_x_96_Inches:16
- Flush:117 (-6.35 mm): Siding_For_Left_Wall:1 ↔ OSB_For_Walls_With_Dimensions_48_x_96_Inches:16
- Mate:134: Siding_For_Left_Wall:1 ↔ Fascia_For_Back:1
- Mate:135 (1.5875 mm): Siding_For_Right_Wall:1 ↔ OSB_For_Walls_With_Dimensions_48_x_96_Inches:17
- Mate:136: Siding_For_Right_Wall:1 ↔ Fascia_For_Back:3
- Flush:118 (-6.35 mm): Siding_For_Right_Wall:1 ↔ OSB_For_Walls_With_Dimensions_37_x_48_Inches:2
- Mate:137 (3.175 mm): Drip_Edge_For_Back:1 ↔ OSB_For_Rear_Roof:2
- Mate:138: Drip_Edge_For_Front:1 ↔ Fascia_For_Front:1
- Flush:119 (-12.7 mm): Drip_Edge_For_Front:1 ↔ Fascia_For_Front:1
- Mate:140: Drip_Edge_For_Side:1 ↔ OSB_For_Rear_Roof:1
- Mate:141: Fascia_For_Side:1 ↔ Drip_Edge_For_Side:1
- Flush:120 (-22.225 mm): Drip_Edge_For_Side:1 ↔ OSB_For_Rear_Roof:1
- Mate:142: Fascia_For_Side:1 ↔ Fascia_For_Back:1
- Mate:144: Underlayment_For_Side:1 ↔ OSB_For_Side_And_Top:1
- Flush:122: Underlayment_For_Side:1 ↔ OSB_For_Walls_With_Dimensions_37_x_48_Inches:1
- Flush:123: Underlayment_For_Side:1 ↔ OSB_For_Side_And_Top:1
- Flush:124: Underlayment_For_Side:2 ↔ Truss:2
- Mate:145: Underlayment_For_Side:2 ↔ OSB_For_Side_And_Top:2
- Flush:125: Underlayment_For_Side:2 ↔ OSB_For_Walls_With_Dimensions_48_x_96_Inches:8
- Mate:146: Underlayment_For_Front:1 ↔ OSB_For_Walls_With_Dimensions_48_x_96_Inches:15
- Flush:126: Underlayment_For_Front:1 ↔ Underlayment_For_Side:2
- Mate:147: Underlayment_For_Front:1 ↔ Truss:2
- Mate:148: OSB_For_Side_And_Top:2 ↔ OSB_For_Roof_With_Dimensions_48_x_48:1
- Mate:149: Truss:19 ↔ OSB_For_Roof_With_Dimensions_48_x_48:1
- Mate:150: OSB_For_Rear_Roof:3 ↔ OSB_For_Roof_With_Dimensions_48_x_48:1
- Mate:151: OSB_For_Rear_Roof:3 ↔ OSB_For_Roof_With_Dimensions_96_x_48:4
- Mate:152: OSB_For_Roof_With_Dimensions_48_x_48:1 ↔ OSB_For_Roof_With_Dimensions_46.416_x_96:1
- Mate:153: Truss:1 ↔ OSB_For_Roof_With_Dimensions_46.416_x_96:1
- Flush:127: Truss:2 ↔ OSB_For_Roof_With_Dimensions_46.416_x_96:1
- Flush:128: OSB_For_Side_And_Back:1 ↔ OSB_For_Rear_Roof:1
